# Autodesk Inventor assembly: Line Sensor Attachment Assembly
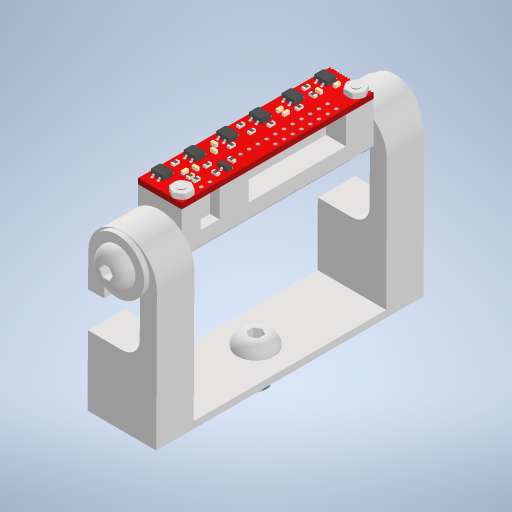
[picture p0: Inventor's stored thumbnail of the model, 512x512]
Saved by Autodesk Inventor 2024 (Build 280153000, 153)
## iProperties
Created: 2023-10-22
Part Number: Line Sensor Attachment Assembly
Document SubType Name: Assembly
Designer: olson
Author: olson
## Documents named in this file (8)
- C:\Users\olson\OneDrive\Documents\Senior Year\FALL 2023\ECE 4961 - Capstone 1\Detial Design\Attachments\CAD\Line Sensor 6 Attachment Assembly.iam
- C:\Users\olson\OneDrive\Documents\Senior Year\FALL 2023\ECE 4961 - Capstone 1\Detial Design\Attachments\CAD\Line Sensor 6 Bracket.ipt
- C:\Users\olson\OneDrive\Documents\Senior Year\FALL 2023\ECE 4961 - Capstone 1\Detial Design\Attachments\CAD\6 Backet Adjustment.ipt
- C:\Users\olson\OneDrive\Documents\Senior Year\FALL 2023\ECE 4961 - Capstone 1\Detial Design\Attachments\CAD\qtr-6rc-reflectance-sensor-array.ipt
- C:\Users\olson\OneDrive\Documents\Senior Year\FALL 2023\ECE 4961 - Capstone 1\Detial Design\Attachments\CAD\1-4 washer.ipt
- C:\Users\olson\OneDrive\Documents\Senior Year\FALL 2023\ECE 4961 - Capstone 1\Detial Design\Attachments\CAD\1-4-20 screw.ipt
- C:\Users\olson\OneDrive\Documents\Senior Year\FALL 2023\ECE 4961 - Capstone 1\Detial Design\Attachments\CAD\2-56 screw.ipt
- C:\Users\olson\OneDrive\Documents\Senior Year\FALL 2023\ECE 4961 - Capstone 1\Detial Design\Attachments\CAD\2-56 nut.ipt
## Components (12 placed, 7 different names)
1. Line Sensor 6 Bracket:1 — Flush:1, Flush:2, Mate:1, Insert:1, Rotational:1, Rotational:2, Rotational:8, Rotational:9
2. 6 Backet Adjustment:1 — Insert:1, Rotational:5
3. qtr-6rc-reflectance-sensor-array:1 — Flush:1, Flush:2, Mate:1, Rotational:7, Rotational:10
4. 1-4-20 screw:1 — Rotational:3
5. 1-4-20 screw:2 — Rotational:4
6. 1-4-20 screw:3 — Rotational:5
7. 1-4 washer:1 — Rotational:1, Rotational:3
8. 1-4 washer:2 — Rotational:2, Rotational:4
9. 2-56 screw:1 — Rotational:9
10. 2-56 screw:2 — Rotational:8
11. 2-56 nut:1 — Rotational:7
12. 2-56 nut:2 — Rotational:10
## Relationships (13: RevoluteJoint 9, Flush 2, Mate 1, Insert 1)
- Flush:1: Line Sensor 6 Bracket:1 ↔ qtr-6rc-reflectance-sensor-array:1
- Flush:2: Line Sensor 6 Bracket:1 ↔ qtr-6rc-reflectance-sensor-array:1
- Mate:1: Line Sensor 6 Bracket:1 ↔ qtr-6rc-reflectance-sensor-array:1
- Insert:1: Line Sensor 6 Bracket:1 ↔ 6 Backet Adjustment:1
- Rotational:1 [RevoluteJoint]: Line Sensor 6 Bracket:1 ↔ 1-4 washer:1
- Rotational:2 [RevoluteJoint]: Line Sensor 6 Bracket:1 ↔ 1-4 washer:2
- Rotational:3 [RevoluteJoint]: 1-4-20 screw:1 ↔ 1-4 washer:1
- Rotational:4 [RevoluteJoint]: 1-4-20 screw:2 ↔ 1-4 washer:2
- Rotational:5 [RevoluteJoint]: 6 Backet Adjustment:1 ↔ 1-4-20 screw:3
- Rotational:7 [RevoluteJoint]: qtr-6rc-reflectance-sensor-array:1 ↔ 2-56 nut:1
- Rotational:8 [RevoluteJoint]: Line Sensor 6 Bracket:1 ↔ 2-56 screw:2
- Rotational:9 [RevoluteJoint]: Line Sensor 6 Bracket:1 ↔ 2-56 screw:1
- Rotational:10 [RevoluteJoint]: qtr-6rc-reflectance-sensor-array:1 ↔ 2-56 nut:2
